# Autodesk Inventor assembly: inner_mirrored
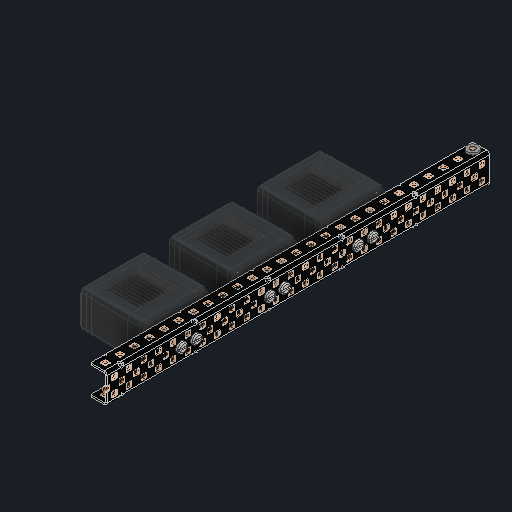
[picture p0: Inventor's stored thumbnail of the model, 512x512]
Saved by Autodesk Inventor 2024 (Build 280153000, 153)
## iProperties
Created: 2024-03-23
Part Number: inner_mirrored
Document SubType Name: Assembly
Designer: Averey Ku
Author: Averey Ku
## Documents named in this file (8)
- D:\vex_robotics\hardware\cad\infection\chassis\mirrored_parts\inner_mirrored.iam
- D:\vex_robotics\hardware\cad\VEX-CAD-Inventor-1.41\Structure\Standoff\Standoff .875.ipt
- D:\vex_robotics\hardware\cad\VEX-CAD-Inventor-1.41\Structure\Standoff.ipt
- D:\vex_robotics\hardware\cad\VEX-CAD-Inventor-1.41\Motion\Spacers\Washer Steel\SWasher .375 OD x .062500.ipt
- D:\vex_robotics\hardware\cad\VEX-CAD-Inventor-1.41\Motion\Spacers\Washer Steel.ipt
- D:\vex_robotics\hardware\cad\infection\chassis\mirrored_parts\V5 Motor_mirrored.ipt
- D:\vex_robotics\hardware\cad\infection\chassis\mirrored_parts\Nylon Screw Pan-Head .500_mirrored.ipt
- D:\vex_robotics\hardware\cad\infection\chassis\mirrored_parts\Alu C 1x2x1x26_mirrored.ipt
## Components (12 placed, 5 different names)
1. Standoff .875:1 — Insert:10
2. SWasher .375 OD x .062500:1 — Insert:9
3. V5 Motor_mirrored:1 — Insert:4, Insert:3
4. Nylon Screw Pan-Head .500_mirrored:1 — Insert:4, Mate:3
5. Nylon Screw Pan-Head .500_mirrored:2 — Insert:3, Insert:13
6. V5 Motor_mirrored:2 — Insert:6, Insert:5
7. Nylon Screw Pan-Head .500_mirrored:3 — Insert:6, Insert:11
8. Nylon Screw Pan-Head .500_mirrored:4 — Insert:5, Mate:1
9. V5 Motor_mirrored:3 — Insert:8, Insert:7
10. Nylon Screw Pan-Head .500_mirrored:5 — Insert:8, Insert:12
11. Nylon Screw Pan-Head .500_mirrored:6 — Insert:7, Mate:2
12. Alu C 1x2x1x26_mirrored:1 — Mate:3, Insert:13, Mate:2, Insert:12, Mate:1, Insert:11, Insert:10, Insert:9
## Relationships (14: Insert 11, Mate 3)
- Insert:4 (1.5875 mm): V5 Motor_mirrored:1 ↔ Nylon Screw Pan-Head .500_mirrored:1
- Insert:3 (1.5875 mm): V5 Motor_mirrored:1 ↔ Nylon Screw Pan-Head .500_mirrored:2
- Insert:6 (1.5875 mm): V5 Motor_mirrored:2 ↔ Nylon Screw Pan-Head .500_mirrored:3
- Insert:5 (1.5875 mm): V5 Motor_mirrored:2 ↔ Nylon Screw Pan-Head .500_mirrored:4
- Insert:8 (1.5875 mm): V5 Motor_mirrored:3 ↔ Nylon Screw Pan-Head .500_mirrored:5
- Insert:7 (1.5875 mm): V5 Motor_mirrored:3 ↔ Nylon Screw Pan-Head .500_mirrored:6
- Mate:3: Nylon Screw Pan-Head .500_mirrored:1 ↔ Alu C 1x2x1x26_mirrored:1
- Insert:13: Nylon Screw Pan-Head .500_mirrored:2 ↔ Alu C 1x2x1x26_mirrored:1
- Mate:2: Nylon Screw Pan-Head .500_mirrored:6 ↔ Alu C 1x2x1x26_mirrored:1
- Insert:12: Nylon Screw Pan-Head .500_mirrored:5 ↔ Alu C 1x2x1x26_mirrored:1
- Mate:1: Nylon Screw Pan-Head .500_mirrored:4 ↔ Alu C 1x2x1x26_mirrored:1
- Insert:11: Nylon Screw Pan-Head .500_mirrored:3 ↔ Alu C 1x2x1x26_mirrored:1
- Insert:10: Standoff .875:1 ↔ Alu C 1x2x1x26_mirrored:1
- Insert:9: SWasher .375 OD x .062500:1 ↔ Alu C 1x2x1x26_mirrored:1
